# Autodesk Inventor assembly: Nexus-pcb
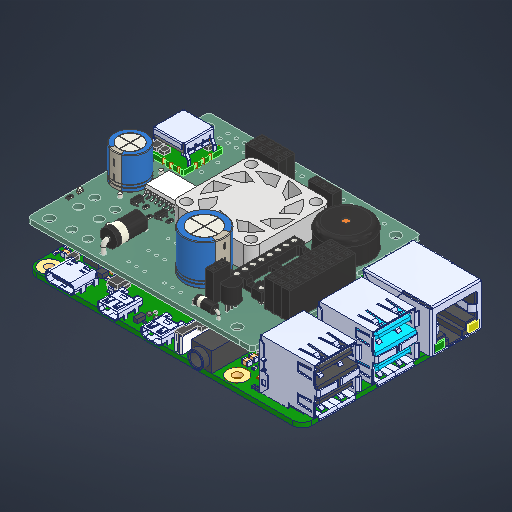
[picture p0: Inventor's stored thumbnail of the model, 512x512]
Saved by Autodesk Inventor 2026.1 (Build 301233020, 233B)
## iProperties
Created: 2026-03-17
Part Number: Nexus-pcb
Document SubType Name: Assembly
Designer: kamada
Author: kamada
## Documents named in this file (3)
- D:\KiCad\KiProject\Nexus\Nexus-3dmodel\Nexus-pcb.iam
- D:\KiCad\KiProject\Nexus\Nexus-3dmodel\Nexus\Nexus\Nexus.iam
- D:\KiCad\KiProject\Nexus\Nexus-3dmodel\Fan.ipt
## Components (2 placed, 2 different names)
1. Nexus:1 [sub-assembly] — 回転:1, 角度:1
2. Fan:1 — 回転:1, 角度:1
## Relationships (2: RevoluteJoint 1, Angle 1)
- 回転:1 [RevoluteJoint]: Nexus:1 ↔ Fan:1
- 角度:1 [Angle] (0 deg): Nexus:1 ↔ Fan:1
